# Autodesk Inventor assembly: Arm
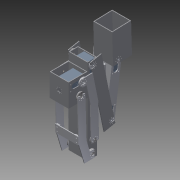
[picture p0: Inventor's stored thumbnail of the model, 180x180]
Saved by Autodesk Inventor 2013 (Build 170138000, 138)
## iProperties
Created: 2014-04-08
Part Number: Arm
Document SubType Name: Assembly
Designer: andou
Author: andou
## Documents named in this file (16)
- C:\Users\andou\Documents\GitHub\Robotics-Project\design\RoboticsProject\project_4\Arm.iam
- C:\Users\andou\Documents\GitHub\Robotics-Project\design\RoboticsProject\project_4\Generic Parts\KRS-2542HV.ipt
- C:\Users\andou\Documents\GitHub\Robotics-Project\design\RoboticsProject\project_4\Generic Parts\Low_Height_Horn.ipt
- C:\Users\andou\Documents\GitHub\Robotics-Project\design\RoboticsProject\project_4\Complete_data\Free_Horn.iam
- C:\Users\andou\Documents\GitHub\Robotics-Project\design\RoboticsProject\project_4\Arm_Bracket.ipt
- C:\Users\andou\Documents\GitHub\Robotics-Project\design\RoboticsProject\project_4\Complete_data\idwなし\First_Link_Flame_4.ipt
- C:\Users\andou\Documents\GitHub\Robotics-Project\design\RoboticsProject\project_4\Complete_data\idwなし\First_Link_Flame_2.ipt
- C:\Users\andou\Documents\GitHub\Robotics-Project\design\RoboticsProject\project_4\Complete_data\Parallel_Link_Supporter.ipt
- C:\Users\andou\Documents\GitHub\Robotics-Project\design\RoboticsProject\project_4\Complete_data\Horn_Spacer.ipt
- C:\Users\andou\Documents\GitHub\Robotics-Project\design\RoboticsProject\project_4\Arm_Second_Flame.ipt
- C:\Users\andou\Documents\GitHub\Robotics-Project\design\RoboticsProject\project_4\Arm_Third_Flame.ipt
- C:\Users\andou\Documents\GitHub\Robotics-Project\design\RoboticsProject\project_4\Complete_data\idwなし\First_Link_Flame_1.ipt
- C:\Users\andou\Documents\GitHub\Robotics-Project\design\RoboticsProject\project_4\Complete_data\idwなし\First_Link_Flame_3.ipt
- C:\Users\andou\Documents\GitHub\Robotics-Project\design\RoboticsProject\project_4\Arm_Fourth_Flame.ipt
- C:\Users\andou\Documents\GitHub\Robotics-Project\design\RoboticsProject\project_4\Third_Flame_Spacer.ipt
- C:\Users\andou\Documents\GitHub\Robotics-Project\design\RoboticsProject\project_4\Arm_Fifth_Flame.ipt
## Components (30 placed, 15 different names)
1. Arm_Bracket:1 — 挿入:2, 挿入:3, 挿入:4, 挿入:14, 挿入:15
2. KRS-2542HV:1 — 挿入:1, 挿入:2, 挿入:3
3. Low_Height_Horn:1 — 挿入:1, 挿入:17, 挿入:18, 挿入:42
4. Free_Horn:1 [sub-assembly] — 挿入:4, 挿入:44
5. Free_Horn:2 [sub-assembly] — 挿入:15, 挿入:45
6. Free_Horn:3 [sub-assembly] — 挿入:14, 挿入:43
7. First_Link_Flame_4:2 — 挿入:8, 挿入:12, 挿入:45
8. First_Link_Flame_2:2 — 挿入:7, 挿入:11, 挿入:25, 挿入:43
9. Parallel_Link_Supporter:2 — 挿入:7, 挿入:8, 挿入:11, 挿入:12
10. Horn_Spacer:1 — 挿入:17, 挿入:18
11. Arm_Second_Flame:1 — 挿入:20, 挿入:21, 挿入:22, 挿入:23, 挿入:26, 挿入:27, 挿入:29
12. Free_Horn:4 [sub-assembly] — 挿入:20
13. Free_Horn:5 [sub-assembly] — 挿入:21, 挿入:41
14. Free_Horn:6 [sub-assembly] — 挿入:23, 挿入:39
15. Free_Horn:7 [sub-assembly] — 挿入:22, 挿入:25
16. Free_Horn:8 [sub-assembly] — 挿入:29, 挿入:46
17. KRS-2542HV:2 — 挿入:26, 挿入:27, 挿入:28
18. Low_Height_Horn:2 — 挿入:28, 挿入:47
19. Arm_Third_Flame:1 — 挿入:46, 挿入:47, 挿入:56, 挿入:57, 挿入:58, 挿入:59
20. First_Link_Flame_1:1 — 挿入:39, 挿入:42
21. First_Link_Flame_3:1 — 挿入:41, 挿入:44
22. Arm_Fourth_Flame:1 — 挿入:48, 挿入:49, 挿入:50, 挿入:51, 挿入:54, 挿入:55
23. KRS-2542HV:3 — 挿入:50, 挿入:51, 挿入:52
24. KRS-2542HV:4 — 挿入:48, 挿入:49, 挿入:53
25. Low_Height_Horn:3 — 挿入:53, 挿入:60
26. Low_Height_Horn:4 — 挿入:52, 挿入:57
27. Free_Horn:9 [sub-assembly] — 挿入:55, 挿入:56
28. Free_Horn:10 [sub-assembly] — 挿入:54
29. Third_Flame_Spacer:1 — 挿入:58, 挿入:59
30. Arm_Fifth_Flame:1 — 挿入:60
## Relationships (42: Insert 42)
- 挿入:1 [Insert]: KRS-2542HV:1 ↔ Low_Height_Horn:1
- 挿入:2 [Insert]: Arm_Bracket:1 ↔ KRS-2542HV:1
- 挿入:3 [Insert]: Arm_Bracket:1 ↔ KRS-2542HV:1
- 挿入:4 [Insert]: Arm_Bracket:1 ↔ Free_Horn:1
- 挿入:7 [Insert]: First_Link_Flame_2:2 ↔ Parallel_Link_Supporter:2
- 挿入:8 [Insert]: First_Link_Flame_4:2 ↔ Parallel_Link_Supporter:2
- 挿入:11 [Insert]: First_Link_Flame_2:2 ↔ Parallel_Link_Supporter:2
- 挿入:12 [Insert]: First_Link_Flame_4:2 ↔ Parallel_Link_Supporter:2
- 挿入:14 [Insert]: Arm_Bracket:1 ↔ Free_Horn:3
- 挿入:15 [Insert]: Arm_Bracket:1 ↔ Free_Horn:2
- 挿入:17 [Insert]: Low_Height_Horn:1 ↔ Horn_Spacer:1
- 挿入:18 [Insert]: Low_Height_Horn:1 ↔ Horn_Spacer:1
- 挿入:20 [Insert]: Arm_Second_Flame:1 ↔ Free_Horn:4
- 挿入:21 [Insert]: Arm_Second_Flame:1 ↔ Free_Horn:5
- 挿入:22 [Insert]: Arm_Second_Flame:1 ↔ Free_Horn:7
- 挿入:23 [Insert]: Arm_Second_Flame:1 ↔ Free_Horn:6
- 挿入:25 [Insert]: First_Link_Flame_2:2 ↔ Free_Horn:7
- 挿入:26 [Insert]: Arm_Second_Flame:1 ↔ KRS-2542HV:2
- 挿入:27 [Insert]: Arm_Second_Flame:1 ↔ KRS-2542HV:2
- 挿入:28 [Insert]: KRS-2542HV:2 ↔ Low_Height_Horn:2
- 挿入:29 [Insert]: Arm_Second_Flame:1 ↔ Free_Horn:8
- 挿入:39 [Insert]: Free_Horn:6 ↔ First_Link_Flame_1:1
- 挿入:41 [Insert]: Free_Horn:5 ↔ First_Link_Flame_3:1
- 挿入:42 [Insert]: Low_Height_Horn:1 ↔ First_Link_Flame_1:1
- 挿入:43 [Insert]: Free_Horn:3 ↔ First_Link_Flame_2:2
- 挿入:44 [Insert]: Free_Horn:1 ↔ First_Link_Flame_3:1
- 挿入:45 [Insert]: Free_Horn:2 ↔ First_Link_Flame_4:2
- 挿入:46 [Insert]: Free_Horn:8 ↔ Arm_Third_Flame:1
- 挿入:47 [Insert]: Low_Height_Horn:2 ↔ Arm_Third_Flame:1
- 挿入:48 [Insert]: Arm_Fourth_Flame:1 ↔ KRS-2542HV:4
- 挿入:49 [Insert]: Arm_Fourth_Flame:1 ↔ KRS-2542HV:4
- 挿入:50 [Insert]: Arm_Fourth_Flame:1 ↔ KRS-2542HV:3
- 挿入:51 [Insert]: Arm_Fourth_Flame:1 ↔ KRS-2542HV:3
- 挿入:52 [Insert]: KRS-2542HV:3 ↔ Low_Height_Horn:4
- 挿入:53 [Insert]: KRS-2542HV:4 ↔ Low_Height_Horn:3
- 挿入:54 [Insert]: Arm_Fourth_Flame:1 ↔ Free_Horn:10
- 挿入:55 [Insert]: Arm_Fourth_Flame:1 ↔ Free_Horn:9
- 挿入:56 [Insert]: Arm_Third_Flame:1 ↔ Free_Horn:9
- 挿入:57 [Insert]: Arm_Third_Flame:1 ↔ Low_Height_Horn:4
- 挿入:58 [Insert]: Arm_Third_Flame:1 ↔ Third_Flame_Spacer:1
- 挿入:59 [Insert]: Arm_Third_Flame:1 ↔ Third_Flame_Spacer:1
- 挿入:60 [Insert]: Low_Height_Horn:3 ↔ Arm_Fifth_Flame:1
